# Autodesk Inventor assembly: motor
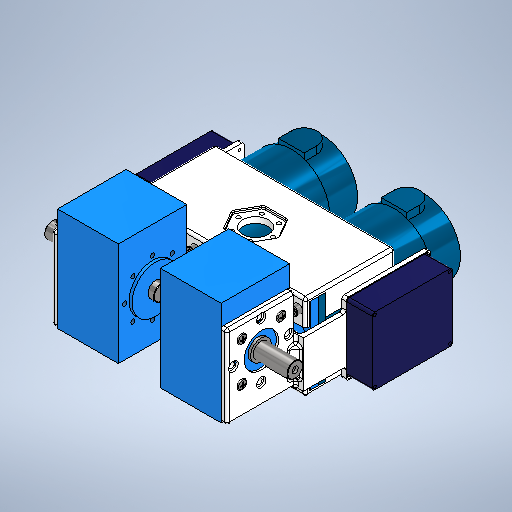
[picture p0: Inventor's stored thumbnail of the model, 512x512]
Saved by Autodesk Inventor 2025.3 (Build 293356030, 356C)
## iProperties
Created: 2025-09-06
Part Number: motor
Document SubType Name: Assembly
Designer: MSI
Mass: 13635.5 g
Surface Area: 5600.72 cm^2
Volume: 4817.73 cm^3
Density: 2.83028 g/cm^3
Author: MSI
## Documents named in this file (10)
- C:\Users\MSI\Desktop\Project\3. 로봇팔\Robot Arm Model\joint4\motor.iam
- C:\Users\MSI\Desktop\Project\3. 로봇팔\Robot Arm Model\joint4\NMRV30_motor.iam
- C:\Users\MSI\Desktop\Project\3. 로봇팔\Robot Arm Model\joint4\motor_holder.ipt
- C:\Users\MSI\Desktop\Project\3. 로봇팔\Robot Arm Model\joint4\motor_shaft.ipt
- C:\Users\MSI\Desktop\Project\3. 로봇팔\Robot Arm Model\joint4\motor_driver.ipt
- C:\Users\MSI\Desktop\Project\3. 로봇팔\Robot Arm Model\joint4\motor_driver_frame_r.ipt
- C:\Users\MSI\Desktop\Project\3. 로봇팔\Robot Arm Model\joint4\motor_driver_frame_l.ipt
- C:\Users\MSI\Documents\Inventor\Content Center Files\R2025\ko-KR\ISO 4762(2)\ISO 4762 - M6 x 30ISO.ipt
- C:\Users\MSI\Documents\Inventor\Content Center Files\R2025\ko-KR\ISO 4032(2)\ISO 4032 - M6 - ISO.ipt
- C:\Users\MSI\Documents\Inventor\Content Center Files\R2025\ko-KR\KS B 1023  H (2)\KS B 1023 - A  M 6 x 8 - H(1).ipt
## Components (30 placed, 9 different names)
1. NMRV30_motor:1 [sub-assembly] — 강체:1, 강체:3, 회전:2, 강체:8, 메이트:2
2. NMRV30_motor:2 [sub-assembly] — 강체:2, 강체:4, 회전:1, 강체:9, 메이트:1
3. motor_holder:1 — 강체:1, 강체:2, 삽입:1, 삽입:2, 삽입:3, 삽입:4, 각도:1, 각도:2, 메이트:3, 메이트:4
4. motor_holder:2 — 강체:3, 강체:4, 삽입:5, 삽입:6, 삽입:7, 삽입:8, 각도:3, 각도:4
5. motor_shaft:1 — 회전:1
6. motor_shaft:2 — 회전:2
7. motor_driver:1 — 강체:6
8. motor_driver:2 — 강체:7
9. motor_driver_frame_r:1 — 강체:8, 강체:7, 삽입:25, 삽입:26, 삽입:27, 삽입:28
10. motor_driver_frame_l:1 — 강체:9, 강체:6, 삽입:21, 삽입:22, 삽입:23, 삽입:24
11. ISO 4762 M6 x 30:1 — 삽입:4
12. ISO 4762 M6 x 30:2 — 삽입:5
13. ISO 4762 M6 x 30:3 — 삽입:3, 삽입:9
14. ISO 4762 M6 x 30:4 — 삽입:6, 삽입:12
15. ISO 4762 M6 x 30:5 — 삽입:8
16. ISO 4762 M6 x 30:6 — 삽입:1
17. ISO 4762 M6 x 30:7 — 삽입:7, 삽입:11
18. ISO 4762 M6 x 30:8 — 삽입:2, 삽입:10
19. ISO 4032 M6:1 — 삽입:12, 각도:4
20. ISO 4032 M6:2 — 삽입:9, 각도:1
21. ISO 4032 M6:3 — 삽입:11, 각도:3
22. ISO 4032 M6:4 — 삽입:10, 각도:2
23. KS B 1023 H - 미터 A  M 6 x 8 - H:1 — 삽입:21
24. KS B 1023 H - 미터 A  M 6 x 8 - H:2 — 삽입:24
25. KS B 1023 H - 미터 A  M 6 x 8 - H:3 — 삽입:23
26. KS B 1023 H - 미터 A  M 6 x 8 - H:4 — 삽입:22
27. KS B 1023 H - 미터 A  M 6 x 8 - H:5 — 삽입:27
28. KS B 1023 H - 미터 A  M 6 x 8 - H:6 — 삽입:28
29. KS B 1023 H - 미터 A  M 6 x 8 - H:7 — 삽입:26
30. KS B 1023 H - 미터 A  M 6 x 8 - H:8 — 삽입:25
## Relationships (38: Insert 20, WeldJoint 8, Mate 4, Angle 4, RevoluteJoint 2)
- 강체:1 [WeldJoint]: NMRV30_motor:1 ↔ motor_holder:1
- 강체:2 [WeldJoint]: NMRV30_motor:2 ↔ motor_holder:1
- 강체:3 [WeldJoint]: NMRV30_motor:1 ↔ motor_holder:2
- 강체:4 [WeldJoint]: NMRV30_motor:2 ↔ motor_holder:2
- 회전:1 [RevoluteJoint]: NMRV30_motor:2 ↔ motor_shaft:1
- 회전:2 [RevoluteJoint]: NMRV30_motor:1 ↔ motor_shaft:2
- 강체:6 [WeldJoint]: motor_driver:1 ↔ motor_driver_frame_l:1
- 강체:7 [WeldJoint]: motor_driver:2 ↔ motor_driver_frame_r:1
- 강체:8 [WeldJoint]: NMRV30_motor:1 ↔ motor_driver_frame_r:1
- 강체:9 [WeldJoint]: NMRV30_motor:2 ↔ motor_driver_frame_l:1
- 메이트:1 [Mate]: NMRV30_motor:2
- 삽입:1 [Insert]: motor_holder:1 ↔ ISO 4762 M6 x 30:6
- 삽입:2 [Insert]: motor_holder:1 ↔ ISO 4762 M6 x 30:8
- 삽입:3 [Insert]: motor_holder:1 ↔ ISO 4762 M6 x 30:3
- 삽입:4 [Insert]: motor_holder:1 ↔ ISO 4762 M6 x 30:1
- 삽입:5 [Insert]: motor_holder:2 ↔ ISO 4762 M6 x 30:2
- 삽입:6 [Insert]: motor_holder:2 ↔ ISO 4762 M6 x 30:4
- 삽입:7 [Insert]: motor_holder:2 ↔ ISO 4762 M6 x 30:7
- 삽입:8 [Insert]: motor_holder:2 ↔ ISO 4762 M6 x 30:5
- 삽입:9 [Insert] (-6.5 mm): ISO 4762 M6 x 30:3 ↔ ISO 4032 M6:2
- 각도:1 [Angle] (0 deg): motor_holder:1 ↔ ISO 4032 M6:2
- 삽입:10 [Insert] (-6.5 mm): ISO 4762 M6 x 30:8 ↔ ISO 4032 M6:4
- 각도:2 [Angle] (0 deg): motor_holder:1 ↔ ISO 4032 M6:4
- 삽입:11 [Insert] (-6.5 mm): ISO 4762 M6 x 30:7 ↔ ISO 4032 M6:3
- 각도:3 [Angle] (0 deg): motor_holder:2 ↔ ISO 4032 M6:3
- 삽입:12 [Insert] (-6.5 mm): ISO 4762 M6 x 30:4 ↔ ISO 4032 M6:1
- 각도:4 [Angle] (0 deg): motor_holder:2 ↔ ISO 4032 M6:1
- 삽입:21 [Insert]: motor_driver_frame_l:1 ↔ KS B 1023 H - 미터 A  M 6 x 8 - H:1
- 메이트:2 [Mate]: NMRV30_motor:1
- 메이트:3 [Mate]: motor_holder:1
- 메이트:4 [Mate]: motor_holder:1
- 삽입:22 [Insert]: motor_driver_frame_l:1 ↔ KS B 1023 H - 미터 A  M 6 x 8 - H:4
- 삽입:23 [Insert]: motor_driver_frame_l:1 ↔ KS B 1023 H - 미터 A  M 6 x 8 - H:3
- 삽입:24 [Insert]: motor_driver_frame_l:1 ↔ KS B 1023 H - 미터 A  M 6 x 8 - H:2
- 삽입:25 [Insert]: motor_driver_frame_r:1 ↔ KS B 1023 H - 미터 A  M 6 x 8 - H:8
- 삽입:26 [Insert]: motor_driver_frame_r:1 ↔ KS B 1023 H - 미터 A  M 6 x 8 - H:7
- 삽입:27 [Insert]: motor_driver_frame_r:1 ↔ KS B 1023 H - 미터 A  M 6 x 8 - H:5
- 삽입:28 [Insert]: motor_driver_frame_r:1 ↔ KS B 1023 H - 미터 A  M 6 x 8 - H:6
